# Autodesk Inventor assembly: Gyrodesignv2editneeded
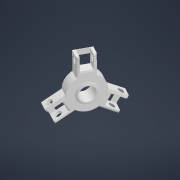
[picture p0: Inventor's stored thumbnail of the model, 180x180]
Saved by Autodesk Inventor 2022 (Build 260153000, 153)
## iProperties
Created: 2021-12-10
Part Number: Gyrodesignv2editneeded
Document SubType Name: Assembly
Designer: Wilson
Author: Wilson
## Documents named in this file (3)
- C:\Users\Wilson\OneDrive\Documents\Projekts\Rocketery\CAD Files v1\Rocoverey System Gyro\Aerospace\Current\Gyrodesignv2editneeded - Copy.iam
- C:\Users\Wilson\OneDrive\Documents\Projekts\Rocketery\CAD Files v1\Rocoverey System Gyro\Aerospace\Current\Gyrocopter Base.ipt
- C:\Users\Wilson\OneDrive\Documents\Projekts\Rocketery\CAD Files v1\Rocoverey System Gyro\Aerospace\Current\Gyrocopter Blade.ipt
## Components (4 placed, 2 different names)
1. Gyrocopter Base:1 — Mate:1, Mate:2, Mate:3
2. Gyrocopter Blade:1 — Mate:1
3. Gyrocopter Blade:3 — Mate:3
4. Gyrocopter Blade:4 — Mate:2
## Relationships (3: Mate 3)
- Mate:1: Gyrocopter Base:1 ↔ Gyrocopter Blade:1
- Mate:2: Gyrocopter Base:1 ↔ Gyrocopter Blade:4
- Mate:3: Gyrocopter Base:1 ↔ Gyrocopter Blade:3
